# Autodesk Inventor assembly: printer
(part 2 of 2)
- Mate:166: z_motor_mount:2 ↔ CSN 02 1702 B B 4,3:122
- Mate:167: z_motor_mount:2 ↔ CSN 02 1702 B B 4,3:122
- Mate:168: frame:1 ↔ CSN 02 1702 B B 4,3:123
- Mate:169: frame:1 ↔ CSN 02 1702 B B 4,3:123
- Mate:170: frame:1 ↔ CSN 02 1702 B B 4,3:124
- Mate:171: frame:1 ↔ CSN 02 1702 B B 4,3:124
- Mate:172: frame:1 ↔ CSN 02 1702 B B 4,3:117
- Mate:173: frame:1 ↔ CSN 02 1702 B B 4,3:117
- Insert:23: CSN 02 1702 B B 4,3:120 ↔ ISO 4762 M4 x 20:64
- Insert:24: CSN 02 1702 B B 4,3:121 ↔ ISO 4762 M4 x 20:63
- Insert:25: CSN 02 1702 B B 4,3:116 ↔ ISO 4762 M4 x 20:62
- Insert:26: CSN 02 1702 B B 4,3:122 ↔ ISO 4762 M4 x 20:61
- Insert:27: CSN 02 1702 B B 4,3:123 ↔ ISO 4762 M4 x 20:60
- Insert:28: CSN 02 1702 B B 4,3:124 ↔ ISO 4762 M4 x 20:58
- Insert:29: CSN 02 1702 B B 4,3:117 ↔ ISO 4762 M4 x 20:59
- Mate:174: z_motor_brace:2 ↔ CSN 02 1702 B B 4,3:125
- Mate:175: CSN 02 1702 B B 4,3:125 ↔ ISO 4762 M4 x 20:59
- Mate:176: z_motor_brace:2 ↔ CSN 02 1702 B B 4,3:115
- Mate:177: CSN 02 1702 B B 4,3:115 ↔ ISO 4762 M4 x 20:64
- Mate:178: z_rod_stopper_bottom:2 ↔ CSN 02 1702 B B 4,3:119
- Mate:179: CSN 02 1702 B B 4,3:119 ↔ ISO 4762 M4 x 20:63
- Mate:180: z_motor_mount:2 ↔ CSN 02 1702 B B 4,3:128
- Mate:181: CSN 02 1702 B B 4,3:128 ↔ ISO 4762 M4 x 20:60
- Mate:182: z_motor_mount:2 ↔ CSN 02 1702 B B 4,3:118
- Mate:183: CSN 02 1702 B B 4,3:118 ↔ ISO 4762 M4 x 20:58
- Mate:184: brace_right:1 ↔ CSN 02 1702 B B 4,3:126
- Mate:185: CSN 02 1702 B B 4,3:126 ↔ ISO 4762 M4 x 20:62
- Mate:186: z_rod_stopper_bottom:2 ↔ CSN 02 1702 B B 4,3:127
- Mate:187: CSN 02 1702 B B 4,3:127 ↔ ISO 4762 M4 x 20:61
- Mate:188: CSN 02 1702 B B 4,3:119 ↔ DIN EN ISO 7040 M4:51
- Mate:189: ISO 4762 M4 x 20:63 ↔ DIN EN ISO 7040 M4:51
- Mate:190: CSN 02 1702 B B 4,3:115 ↔ DIN EN ISO 7040 M4:54
- Mate:191: ISO 4762 M4 x 20:64 ↔ DIN EN ISO 7040 M4:54
- Mate:192: CSN 02 1702 B B 4,3:125 ↔ DIN EN ISO 7040 M4:52
- Mate:193: ISO 4762 M4 x 20:59 ↔ DIN EN ISO 7040 M4:52
- Mate:194: CSN 02 1702 B B 4,3:128 ↔ DIN EN ISO 7040 M4:53
- Mate:195: ISO 4762 M4 x 20:60 ↔ DIN EN ISO 7040 M4:53
- Mate:196: CSN 02 1702 B B 4,3:118 ↔ DIN EN ISO 7040 M4:55
- Mate:197: ISO 4762 M4 x 20:58 ↔ DIN EN ISO 7040 M4:55
- Mate:198: CSN 02 1702 B B 4,3:126 ↔ DIN EN ISO 7040 M4:50
- Mate:199: ISO 4762 M4 x 20:62 ↔ DIN EN ISO 7040 M4:50
- Mate:200: CSN 02 1702 B B 4,3:127 ↔ DIN EN ISO 7040 M4:49
- Mate:201: ISO 4762 M4 x 20:61 ↔ DIN EN ISO 7040 M4:49
- Mate:202: brace_right:1 ↔ wiring_brace:1
- Mate:203: frame:1 ↔ wiring_brace:1
- Mate:204: brace_right:1 ↔ wiring_brace:1
- Mate:205: brace_left:1 ↔ wiring_brace:2
- Mate:206: frame:1 ↔ wiring_brace:2
- Mate:207: brace_left:1 ↔ wiring_brace:2
- Mate:208: frame:1 ↔ CSN 02 1702 B B 4,3:132
- Mate:209: frame:1 ↔ CSN 02 1702 B B 4,3:132
- Mate:210: wiring_brace:1 ↔ CSN 02 1702 B B 4,3:131
- Mate:211: brace_right:1 ↔ CSN 02 1702 B B 4,3:129
- Mate:212: brace_right:1 ↔ CSN 02 1702 B B 4,3:129
- Mate:213: wiring_brace:1 ↔ CSN 02 1702 B B 4,3:130
- Insert:30: CSN 02 1702 B B 4,3:132 ↔ ISO 4762 M4 x 20:65
- Insert:31: CSN 02 1702 B B 4,3:129 ↔ ISO 4762 M4 x 20:66
- Mate:214: CSN 02 1702 B B 4,3:131 ↔ ISO 4762 M4 x 20:65
- Mate:215: CSN 02 1702 B B 4,3:130 ↔ ISO 4762 M4 x 20:66
- Mate:216: CSN 02 1702 B B 4,3:131 ↔ DIN EN ISO 7040 M4:57
- Mate:217: ISO 4762 M4 x 20:65 ↔ DIN EN ISO 7040 M4:57
- Mate:218: CSN 02 1702 B B 4,3:130 ↔ DIN EN ISO 7040 M4:56
- Mate:219: ISO 4762 M4 x 20:66 ↔ DIN EN ISO 7040 M4:56
- Mate:220: z_motor_mount:2 ↔ CSN 02 1702 B B 3,2:3
- Mate:221: z_motor_mount:2 ↔ CSN 02 1702 B B 3,2:2
- Mate:222: z_motor_mount:2 ↔ CSN 02 1702 B B 3,2:1
- Mate:223: z_motor_mount:2 ↔ CSN 02 1702 B B 3,2:4
- Mate:224: z_motor_mount:2 ↔ CSN 02 1702 B B 3,2:2
- Mate:225: z_motor_mount:2 ↔ CSN 02 1702 B B 3,2:4
- Mate:226: z_motor_mount:2 ↔ CSN 02 1702 B B 3,2:3
- Mate:227: z_motor_mount:2 ↔ CSN 02 1702 B B 3,2:1
- Insert:32: CSN 02 1702 B B 3,2:4 ↔ ISO 4762 M3 x 16:2
- Insert:33: CSN 02 1702 B B 3,2:2 ↔ ISO 4762 M3 x 16:1
- Insert:34: CSN 02 1702 B B 3,2:3 ↔ ISO 4762 M3 x 16:3
- Insert:35: CSN 02 1702 B B 3,2:1 ↔ ISO 4762 M3 x 16:4
- Mate:228: CSN 02 1702 B B 4,3:136 ↔ ISO 4762 M4 x 20:67
- Insert:36: CSN 02 1702 B B 4,3:142 ↔ ISO 4762 M4 x 20:67
- Mate:229: CSN 02 1702 B B 4,3:143 ↔ ISO 4762 M4 x 20:68
- Insert:37: CSN 02 1702 B B 4,3:135 ↔ ISO 4762 M4 x 20:68
- Mate:230: CSN 02 1702 B B 4,3:146 ↔ ISO 4762 M4 x 20:69
- Insert:38: CSN 02 1702 B B 4,3:141 ↔ ISO 4762 M4 x 20:69
- Mate:231: CSN 02 1702 B B 4,3:145 ↔ ISO 4762 M4 x 20:70
- Insert:39: CSN 02 1702 B B 4,3:140 ↔ ISO 4762 M4 x 20:70
- Mate:232: CSN 02 1702 B B 4,3:144 ↔ ISO 4762 M4 x 20:71
- Insert:40: CSN 02 1702 B B 4,3:134 ↔ ISO 4762 M4 x 20:71
- Mate:233: CSN 02 1702 B B 4,3:137 ↔ ISO 4762 M4 x 20:72
- Insert:41: CSN 02 1702 B B 4,3:139 ↔ ISO 4762 M4 x 20:72
- Mate:234: CSN 02 1702 B B 4,3:133 ↔ ISO 4762 M4 x 20:73
- Insert:42: CSN 02 1702 B B 4,3:138 ↔ ISO 4762 M4 x 20:73
- Mate:235: ISO 4762 M4 x 20:70 ↔ DIN EN ISO 7040 M4:58
- Mate:236: CSN 02 1702 B B 4,3:145 ↔ DIN EN ISO 7040 M4:58
- Mate:237: ISO 4762 M4 x 20:71 ↔ DIN EN ISO 7040 M4:59
- Mate:238: CSN 02 1702 B B 4,3:144 ↔ DIN EN ISO 7040 M4:59
- Mate:239: ISO 4762 M4 x 20:72 ↔ DIN EN ISO 7040 M4:60
- Mate:240: CSN 02 1702 B B 4,3:137 ↔ DIN EN ISO 7040 M4:60
- Mate:241: ISO 4762 M4 x 20:68 ↔ DIN EN ISO 7040 M4:61
- Mate:242: CSN 02 1702 B B 4,3:143 ↔ DIN EN ISO 7040 M4:61
- Mate:243: ISO 4762 M4 x 20:69 ↔ DIN EN ISO 7040 M4:62
- Mate:244: CSN 02 1702 B B 4,3:146 ↔ DIN EN ISO 7040 M4:62
- Mate:245: ISO 4762 M4 x 20:73 ↔ DIN EN ISO 7040 M4:63
- Mate:246: CSN 02 1702 B B 4,3:133 ↔ DIN EN ISO 7040 M4:63
- Mate:247: ISO 4762 M4 x 20:67 ↔ DIN EN ISO 7040 M4:64
- Mate:248: CSN 02 1702 B B 4,3:136 ↔ DIN EN ISO 7040 M4:64
- Mate:249: CSN 02 1702 B B 4,3:149 ↔ ISO 4762 M4 x 20:74
- Insert:43: CSN 02 1702 B B 4,3:150 ↔ ISO 4762 M4 x 20:74
- Mate:250: CSN 02 1702 B B 4,3:148 ↔ ISO 4762 M4 x 20:75
- Insert:44: CSN 02 1702 B B 4,3:147 ↔ ISO 4762 M4 x 20:75
- Mate:251: ISO 4762 M4 x 20:75 ↔ DIN EN ISO 7040 M4:65
- Mate:252: CSN 02 1702 B B 4,3:148 ↔ DIN EN ISO 7040 M4:65
- Mate:253: ISO 4762 M4 x 20:74 ↔ DIN EN ISO 7040 M4:66
- Mate:254: CSN 02 1702 B B 4,3:149 ↔ DIN EN ISO 7040 M4:66
- Insert:45: CSN 02 1702 B B 3,2:6 ↔ ISO 4762 M3 x 16:5
- Insert:46: CSN 02 1702 B B 3,2:8 ↔ ISO 4762 M3 x 16:6
- Insert:47: CSN 02 1702 B B 3,2:7 ↔ ISO 4762 M3 x 16:7
- Insert:48: CSN 02 1702 B B 3,2:5 ↔ ISO 4762 M3 x 16:8
- Mate:255: back:1 ↔ PC Fan:1
- Mate:256: back:1 ↔ PC Fan:1
- Mate:257: back:1 ↔ PC Fan:1
- Mate:258 (3 mm): back:1 ↔ User Library-Fan Guard:1
- Mate:259: y_carriage_belt_iddler:2 ↔ y_carriage_belt_iddler_holder:1
- Mate:260: y_carriage_belt_iddler:2 ↔ y_carriage_belt_iddler_holder:1
- Mate:261: y_carriage_belt_iddler:2 ↔ y_carriage_belt_iddler_holder:1
- Mate:262: y_carriage_belt_iddler:1 ↔ y_carriage_belt_iddler_holder:1
- Mate:263: y_carriage_belt_iddler:1 ↔ y_carriage_belt_iddler_holder:1
- Mate:264: y_carriage_belt_iddler:1 ↔ y_carriage_belt_iddler_holder:1
- Mate:265: 608RS:1 ↔ belt_guide:1
- Mate:266: 608RS:1 ↔ belt_guide:1
- Mate:267: belt_guide:1 ↔ belt_guide:2
- Mate:268: belt_guide:1 ↔ belt_guide:2
- Mate:269: 608RS:1 ↔ belt_guide:2
- Mate:270: CSN 02 1702 B B 8,4:5 ↔ CSN 02 1702 B B 8,4:6
- Mate:271: CSN 02 1702 B B 8,4:5 ↔ CSN 02 1702 B B 8,4:6
- Mate:272: CSN 02 1702 B B 8,4:3 ↔ CSN 02 1702 B B 8,4:4
- Mate:273: CSN 02 1702 B B 8,4:3 ↔ CSN 02 1702 B B 8,4:4
- Mate:274: 608RS:1 ↔ CSN 02 1702 B B 8,4:4
- Mate:275: 608RS:1 ↔ CSN 02 1702 B B 8,4:4
- Mate:276: 608RS:1 ↔ CSN 02 1702 B B 8,4:5
- Mate:277: 608RS:1 ↔ CSN 02 1702 B B 8,4:5
- Mate:278: y_carriage_belt_iddler:1 ↔ CSN 02 1702 B B 8,4:6
- Mate:279: y_carriage_belt_iddler:2 ↔ 608RS:1
- Mate:280: y_carriage_belt_iddler:2 ↔ CSN 02 1702 B B 8,4:1
- Mate:281: y_carriage_belt_iddler:2 ↔ CSN 02 1702 B B 8,4:1
- Mate:282: y_carriage_belt_iddler:1 ↔ CSN 02 1702 B B 8,4:2
- Mate:283: y_carriage_belt_iddler:1 ↔ CSN 02 1702 B B 8,4:2
- Insert:49: CSN 02 1702 B B 8,4:2 ↔ ISO 4762 M8 x 40:1
- Mate:284: CSN 02 1702 B B 8,4:1 ↔ DIN EN ISO 7040 M8:1
- Mate:285: ISO 4762 M8 x 40:1 ↔ DIN EN ISO 7040 M8:1
- Mate:286: back:1 ↔ y_carriage_belt_iddler:2
- Mate:287: back:1 ↔ y_carriage_belt_iddler:2
- Mate:288: back:1 ↔ y_carriage_belt_iddler:1
- Mate:289: back:1 ↔ CSN 02 1702 B B 4,3:152
- Mate:290: back:1 ↔ CSN 02 1702 B B 4,3:153
- Mate:291: back:1 ↔ CSN 02 1702 B B 4,3:153
- Mate:292: back:1 ↔ CSN 02 1702 B B 4,3:152
- Insert:50: CSN 02 1702 B B 4,3:152 ↔ ISO 4762 M4 x 30:1
- Insert:51: CSN 02 1702 B B 4,3:153 ↔ ISO 4762 M4 x 30:2
- Mate:293: y_carriage_belt_iddler_holder:1 ↔ CSN 02 1702 B B 4,3:154
- Mate:294: y_carriage_belt_iddler_holder:1 ↔ CSN 02 1702 B B 4,3:151
- Mate:295: CSN 02 1702 B B 4,3:151 ↔ ISO 4762 M4 x 30:2
- Mate:296: CSN 02 1702 B B 4,3:154 ↔ ISO 4762 M4 x 30:1
- Mate:297: CSN 02 1702 B B 4,3:151 ↔ DIN EN ISO 7040 M4:68
- Mate:298: ISO 4762 M4 x 30:2 ↔ DIN EN ISO 7040 M4:68
- Mate:299: CSN 02 1702 B B 4,3:154 ↔ DIN EN ISO 7040 M4:67
- Mate:300: ISO 4762 M4 x 30:1 ↔ DIN EN ISO 7040 M4:67
- Mate:301: y_motor_mount:1 ↔ y_motor_mount_brace:1
- Mate:302: y_motor_mount:1 ↔ y_motor_mount_brace:1
- Mate:303: y_motor_mount:1 ↔ y_motor_mount_brace:1
- Mate:304: front:1 ↔ y_motor_mount:1
- Mate:305: front:1 ↔ y_motor_mount_brace:1
- Mate:306: front:1 ↔ y_motor_mount:1
- Mate:307: front:1 ↔ CSN 02 1702 B B 4,3:159
- Mate:308: front:1 ↔ CSN 02 1702 B B 4,3:160
- Mate:309: front:1 ↔ CSN 02 1702 B B 4,3:160
- Mate:310: front:1 ↔ CSN 02 1702 B B 4,3:159
- Mate:311: y_motor_mount:1 ↔ CSN 02 1702 B B 4,3:157
- Mate:312: y_motor_mount:1 ↔ CSN 02 1702 B B 4,3:157
- Insert:52: CSN 02 1702 B B 4,3:160 ↔ ISO 4762 M4 x 20:78
- Insert:53: CSN 02 1702 B B 4,3:159 ↔ ISO 4762 M4 x 20:77
- Insert:54: CSN 02 1702 B B 4,3:157 ↔ ISO 4762 M4 x 20:76
- Mate:313: y_motor_mount_brace:1 ↔ CSN 02 1702 B B 4,3:158
- Mate:314: CSN 02 1702 B B 4,3:158 ↔ ISO 4762 M4 x 20:78
- Mate:315: y_motor_mount_brace:1 ↔ CSN 02 1702 B B 4,3:155
- Mate:316: CSN 02 1702 B B 4,3:155 ↔ ISO 4762 M4 x 20:76
- Mate:317: y_motor_mount:1 ↔ CSN 02 1702 B B 4,3:156
- Mate:318: CSN 02 1702 B B 4,3:156 ↔ ISO 4762 M4 x 20:77
- Mate:319: CSN 02 1702 B B 4,3:156 ↔ DIN EN ISO 7040 M4:70
- Mate:320: ISO 4762 M4 x 20:77 ↔ DIN EN ISO 7040 M4:70
- Mate:321: CSN 02 1702 B B 4,3:158 ↔ DIN EN ISO 7040 M4:69
- Mate:322: ISO 4762 M4 x 20:78 ↔ DIN EN ISO 7040 M4:69
- Mate:323: CSN 02 1702 B B 4,3:155 ↔ DIN EN ISO 7040 M4:71
- Mate:324: ISO 4762 M4 x 20:76 ↔ DIN EN ISO 7040 M4:71
- Mate:325: motor_spacer:1 ↔ NEMA 17 with T5 Pulley:1
- Mate:326: motor_spacer:1 ↔ NEMA 17 with T5 Pulley:1
- Mate:327: motor_spacer:1 ↔ NEMA 17 with T5 Pulley:1
- Mate:328: y_motor_mount:1 ↔ motor_spacer:1
- Tangent:1: y_motor_mount:1 ↔ motor_spacer:1
- Tangent:2: y_motor_mount:1 ↔ motor_spacer:1
- Mate:329: y_motor_mount:1 ↔ CSN 02 1702 B B 3,2:12
- Mate:330: y_motor_mount:1 ↔ CSN 02 1702 B B 3,2:11
- Mate:331: y_motor_mount:1 ↔ CSN 02 1702 B B 3,2:9
- Mate:332: y_motor_mount:1 ↔ CSN 02 1702 B B 3,2:10
- Insert:55: CSN 02 1702 B B 3,2:12 ↔ ISO 4762 M3 x 16:12
- Insert:56: CSN 02 1702 B B 3,2:11 ↔ ISO 4762 M3 x 16:11
- Insert:57: CSN 02 1702 B B 3,2:9 ↔ ISO 4762 M3 x 16:10
- Insert:58: CSN 02 1702 B B 3,2:10 ↔ ISO 4762 M3 x 16:9
- Mate:333: motor_spacer:1 ↔ ISO 4762 M3 x 16:12
- Mate:334: motor_spacer:1 ↔ ISO 4762 M3 x 16:11
- Mate:335: motor_spacer:1 ↔ ISO 4762 M3 x 16:9
- Mate:336: motor_spacer:1 ↔ ISO 4762 M3 x 16:10
- Mate:337: y_axis_rod:2 ↔ y_carryage:1
- Mate:338: y_axis_rod:1 ↔ y_carryage:1
- Mate:339: z_axis_rod:2 ↔ x_axis:1
- Mate:340: z_axis_rod:1 ↔ x_axis:1
- Mate:341: brace_right:1 ↔ CSN 02 1702 B B 4,3:161
- Mate:342: brace_right:1 ↔ CSN 02 1702 B B 4,3:161
- Insert:59: CSN 02 1702 B B 4,3:161 ↔ ISO 4762 M4 x 20:79
- Mate:343: frame_brace_top:1 ↔ CSN 02 1702 B B 4,3:162
- Mate:344: CSN 02 1702 B B 4,3:162 ↔ ISO 4762 M4 x 20:79
- Mate:345: CSN 02 1702 B B 4,3:162 ↔ DIN EN ISO 7040 M4:72
- Mate:346: ISO 4762 M4 x 20:79 ↔ DIN EN ISO 7040 M4:72
- Mate:347: CSN 02 1702 B B 4,3:164 ↔ ISO 4762 M4 x 20:80
- Insert:60: CSN 02 1702 B B 4,3:163 ↔ ISO 4762 M4 x 20:80
- Mate:348: ISO 4762 M4 x 20:80 ↔ DIN EN ISO 7040 M4:73
- Mate:349: CSN 02 1702 B B 4,3:164 ↔ DIN EN ISO 7040 M4:73
- Mate:350: z_axis_top_cap:2 ↔ CSN 02 1702 B B 4,3:172
- Mate:351: z_axis_top_cap:2 ↔ CSN 02 1702 B B 4,3:174
- Mate:352: z_axis_top_cap:2 ↔ CSN 02 1702 B B 4,3:174
- Mate:353: z_axis_top_cap:2 ↔ CSN 02 1702 B B 4,3:172
- Mate:354: z_axis_top:2 ↔ CSN 02 1702 B B 4,3:173
- Mate:355: z_axis_top:2 ↔ CSN 02 1702 B B 4,3:171
- Mate:356: z_axis_top:2 ↔ CSN 02 1702 B B 4,3:170
- Mate:357: z_axis_top:2 ↔ CSN 02 1702 B B 4,3:170
- Mate:358: z_axis_top:2 ↔ CSN 02 1702 B B 4,3:173
- Mate:359: z_axis_top:2 ↔ CSN 02 1702 B B 4,3:171
- Insert:61: CSN 02 1702 B B 4,3:170 ↔ ISO 4762 M4 x 20:81
- Insert:62: CSN 02 1702 B B 4,3:171 ↔ ISO 4762 M4 x 20:82
- Insert:63: CSN 02 1702 B B 4,3:173 ↔ ISO 4762 M4 x 20:83
- Insert:64: CSN 02 1702 B B 4,3:174 ↔ ISO 4762 M4 x 20:84
- Insert:65: CSN 02 1702 B B 4,3:172 ↔ ISO 4762 M4 x 20:85
- Mate:360: brace_right:1 ↔ CSN 02 1702 B B 4,3:169
- Mate:361: CSN 02 1702 B B 4,3:169 ↔ ISO 4762 M4 x 20:81
- Mate:362: frame:1 ↔ CSN 02 1702 B B 4,3:165
- Mate:363: CSN 02 1702 B B 4,3:165 ↔ ISO 4762 M4 x 20:83
- Mate:364: frame:1 ↔ CSN 02 1702 B B 4,3:166
- Mate:365: CSN 02 1702 B B 4,3:166 ↔ ISO 4762 M4 x 20:82
- Mate:366: z_axis_top:2 ↔ CSN 02 1702 B B 4,3:167
- Mate:367: CSN 02 1702 B B 4,3:167 ↔ ISO 4762 M4 x 20:84
- Mate:368: z_axis_top:2 ↔ CSN 02 1702 B B 4,3:168
- Mate:369: CSN 02 1702 B B 4,3:169 ↔ DIN EN ISO 7040 M4:78
- Mate:370: ISO 4762 M4 x 20:81 ↔ DIN EN ISO 7040 M4:78
- Mate:371: CSN 02 1702 B B 4,3:166 ↔ DIN EN ISO 7040 M4:77
- Mate:372: ISO 4762 M4 x 20:82 ↔ DIN EN ISO 7040 M4:77
- Mate:373: CSN 02 1702 B B 4,3:165 ↔ DIN EN ISO 7040 M4:76
- Mate:374: ISO 4762 M4 x 20:83 ↔ DIN EN ISO 7040 M4:76
- Mate:375: CSN 02 1702 B B 4,3:167 ↔ DIN EN ISO 7040 M4:75
- Mate:376: ISO 4762 M4 x 20:84 ↔ DIN EN ISO 7040 M4:75
- Mate:377: CSN 02 1702 B B 4,3:168 ↔ DIN EN ISO 7040 M4:74
- Mate:378: CSN 02 1702 B B 4,3:168 ↔ ISO 4762 M4 x 20:85
- Mate:379: ISO 4762 M4 x 20:85 ↔ DIN EN ISO 7040 M4:74
- Mate:380: CSN 02 1702 B B 4,3:179 ↔ ISO 4762 M4 x 20:86
- Insert:66: CSN 02 1702 B B 4,3:180 ↔ ISO 4762 M4 x 20:86
- Mate:381: CSN 02 1702 B B 4,3:176 ↔ ISO 4762 M4 x 20:87
- Insert:67: CSN 02 1702 B B 4,3:181 ↔ ISO 4762 M4 x 20:87
- Mate:382: CSN 02 1702 B B 4,3:175 ↔ ISO 4762 M4 x 20:88
- Insert:68: CSN 02 1702 B B 4,3:183 ↔ ISO 4762 M4 x 20:88
- Mate:383: CSN 02 1702 B B 4,3:177 ↔ ISO 4762 M4 x 20:89
- Insert:69: CSN 02 1702 B B 4,3:184 ↔ ISO 4762 M4 x 20:89
- Mate:384: CSN 02 1702 B B 4,3:178 ↔ ISO 4762 M4 x 20:90
- Insert:70: CSN 02 1702 B B 4,3:182 ↔ ISO 4762 M4 x 20:90
- Mate:385: ISO 4762 M4 x 20:90 ↔ DIN EN ISO 7040 M4:79
- Mate:386: CSN 02 1702 B B 4,3:178 ↔ DIN EN ISO 7040 M4:79
- Mate:387: ISO 4762 M4 x 20:89 ↔ DIN EN ISO 7040 M4:80
- Mate:388: CSN 02 1702 B B 4,3:177 ↔ DIN EN ISO 7040 M4:80
- Mate:389: ISO 4762 M4 x 20:88 ↔ DIN EN ISO 7040 M4:81
- Mate:390: CSN 02 1702 B B 4,3:175 ↔ DIN EN ISO 7040 M4:81
- Mate:391: ISO 4762 M4 x 20:87 ↔ DIN EN ISO 7040 M4:82
- Mate:392: CSN 02 1702 B B 4,3:176 ↔ DIN EN ISO 7040 M4:82
- Mate:393: ISO 4762 M4 x 20:86 ↔ DIN EN ISO 7040 M4:83
- Mate:394: CSN 02 1702 B B 4,3:179 ↔ DIN EN ISO 7040 M4:83
- Mate:402: front:1 ↔ front_panel_2004_brace_left:1
- Mate:403: front:1 ↔ front_panel_2004_brace_left:1
- Flush:7: front:1 ↔ front_panel_2004_brace_left:1
- Flush:8: lcd:1 ↔ front_panel_2004_display:1
- Mate:404: lcd:1 ↔ front_panel_2004_display:1
- Mate:405: lcd:1 ↔ front_panel_2004_display:1
- Mate:406: front_panel_2004_brace_left:1 ↔ front_panel_2004_display:1
- Mate:407: front_panel_2004_brace_left:1 ↔ front_panel_2004_display:1
- Mate:408: front_panel_2004_brace_left:1 ↔ front_panel_2004_display:1
- Mate:409: front_panel_2004_brace_left:1 ↔ front_panel_2004_front:1
- Mate:410: front_panel_2004_brace_left:1 ↔ front_panel_2004_front:1
- Mate:411: front_panel_2004_brace_left:1 ↔ front_panel_2004_front:1
- Mate:412: front_panel_2004_brace_left:1 ↔ front_panel_2004_bottom:1
- Mate:413: front_panel_2004_brace_left:1 ↔ front_panel_2004_bottom:1
- Mate:414: front_panel_2004_brace_left:1 ↔ front_panel_2004_bottom:1
- Mate:415: front:1 ↔ front_panel_2004_brace_right:1
- Mate:416: front_panel_2004_display:1 ↔ front_panel_2004_brace_right:1
- Mate:417: front_panel_2004_display:1 ↔ front_panel_2004_brace_right:1
- Mate:418: front_panel_2004_brace_right:1 ↔ CSN 02 1702 B B 4,3:199
- Mate:419: front_panel_2004_brace_right:1 ↔ CSN 02 1702 B B 4,3:199
- Mate:420: front_panel_2004_brace_right:1 ↔ CSN 02 1702 B B 4,3:200
- Mate:421: front_panel_2004_brace_right:1 ↔ CSN 02 1702 B B 4,3:200
- Mate:422: front_panel_2004_brace_right:1 ↔ CSN 02 1702 B B 4,3:198
- Mate:423: front_panel_2004_brace_right:1 ↔ CSN 02 1702 B B 4,3:198
- Mate:424: front_panel_2004_brace_right:1 ↔ CSN 02 1702 B B 4,3:197
- Mate:425: front_panel_2004_brace_right:1 ↔ CSN 02 1702 B B 4,3:197
- Mate:426: front_panel_2004_brace_right:1 ↔ CSN 02 1702 B B 4,3:196
- Mate:427: front_panel_2004_brace_right:1 ↔ CSN 02 1702 B B 4,3:196
- Mate:428: front_panel_2004_brace_right:1 ↔ CSN 02 1702 B B 4,3:195
- Mate:429: front_panel_2004_brace_right:1 ↔ CSN 02 1702 B B 4,3:195
- Mate:430: front:1 ↔ CSN 02 1702 B B 4,3:194
- Mate:431: front:1 ↔ CSN 02 1702 B B 4,3:194
- Mate:432: front:1 ↔ CSN 02 1702 B B 4,3:186
- Mate:433: front:1 ↔ CSN 02 1702 B B 4,3:186
- Insert:71: CSN 02 1702 B B 4,3:197 ↔ ISO 4762 M4 x 20:91
- Insert:72: CSN 02 1702 B B 4,3:199 ↔ ISO 4762 M4 x 20:98
- Insert:73: CSN 02 1702 B B 4,3:196 ↔ ISO 4762 M4 x 20:97
- Insert:74: CSN 02 1702 B B 4,3:195 ↔ ISO 4762 M4 x 20:92
- Insert:75: CSN 02 1702 B B 4,3:200 ↔ ISO 4762 M4 x 20:93
- Insert:76: CSN 02 1702 B B 4,3:198 ↔ ISO 4762 M4 x 20:94
- Insert:77: CSN 02 1702 B B 4,3:186 ↔ ISO 4762 M4 x 20:95
- Insert:78: CSN 02 1702 B B 4,3:194 ↔ ISO 4762 M4 x 20:96
- Mate:434: front_panel_2004_display:1 ↔ CSN 02 1702 B B 4,3:193
- Mate:435: CSN 02 1702 B B 4,3:193 ↔ ISO 4762 M4 x 20:94
- Mate:436: front_panel_2004_display:1 ↔ CSN 02 1702 B B 4,3:187
- Mate:437: CSN 02 1702 B B 4,3:187 ↔ ISO 4762 M4 x 20:93
- Mate:438: front_panel_2004_display:1 ↔ CSN 02 1702 B B 4,3:188
- Mate:439: CSN 02 1702 B B 4,3:188 ↔ ISO 4762 M4 x 20:98
- Mate:440: front_panel_2004_front:1 ↔ CSN 02 1702 B B 4,3:185
- Mate:441: CSN 02 1702 B B 4,3:185 ↔ ISO 4762 M4 x 20:91
- Mate:442: front_panel_2004_brace_right:1 ↔ CSN 02 1702 B B 4,3:192
- Mate:443: CSN 02 1702 B B 4,3:192 ↔ ISO 4762 M4 x 20:96
- Mate:444: front_panel_2004_brace_right:1 ↔ CSN 02 1702 B B 4,3:189
- Mate:445: CSN 02 1702 B B 4,3:189 ↔ ISO 4762 M4 x 20:95
- Mate:446: front_panel_2004_bottom:1 ↔ CSN 02 1702 B B 4,3:191
- Mate:447: CSN 02 1702 B B 4,3:191 ↔ ISO 4762 M4 x 20:97
- Mate:448: front_panel_2004_bottom:1 ↔ CSN 02 1702 B B 4,3:190
- Mate:449: CSN 02 1702 B B 4,3:190 ↔ ISO 4762 M4 x 20:92
- Mate:450: CSN 02 1702 B B 4,3:190 ↔ DIN EN ISO 7040 M4:91
- Mate:451: ISO 4762 M4 x 20:92 ↔ DIN EN ISO 7040 M4:91
- Mate:452: CSN 02 1702 B B 4,3:191 ↔ DIN EN ISO 7040 M4:85
- Mate:453: ISO 4762 M4 x 20:97 ↔ DIN EN ISO 7040 M4:85
- Mate:454: CSN 02 1702 B B 4,3:185 ↔ DIN EN ISO 7040 M4:84
- Mate:455: ISO 4762 M4 x 20:91 ↔ DIN EN ISO 7040 M4:84
- Mate:456: CSN 02 1702 B B 4,3:188 ↔ DIN EN ISO 7040 M4:90
- Mate:457: ISO 4762 M4 x 20:98 ↔ DIN EN ISO 7040 M4:90
- Mate:458: CSN 02 1702 B B 4,3:187 ↔ DIN EN ISO 7040 M4:89
- Mate:459: ISO 4762 M4 x 20:93 ↔ DIN EN ISO 7040 M4:89
- Mate:460: CSN 02 1702 B B 4,3:193 ↔ DIN EN ISO 7040 M4:86
- Mate:461: ISO 4762 M4 x 20:94 ↔ DIN EN ISO 7040 M4:86
- Mate:462: CSN 02 1702 B B 4,3:192 ↔ DIN EN ISO 7040 M4:87
- Mate:463: ISO 4762 M4 x 20:96 ↔ DIN EN ISO 7040 M4:87
- Mate:464: CSN 02 1702 B B 4,3:189 ↔ DIN EN ISO 7040 M4:88
- Mate:465: ISO 4762 M4 x 20:95 ↔ DIN EN ISO 7040 M4:88
- Mate:466: CSN 02 1702 B B 4,3:201 ↔ ISO 4762 M4 x 20:99
- Insert:79: CSN 02 1702 B B 4,3:211 ↔ ISO 4762 M4 x 20:99
- Mate:467: CSN 02 1702 B B 4,3:205 ↔ ISO 4762 M4 x 20:100
- Insert:80: CSN 02 1702 B B 4,3:209 ↔ ISO 4762 M4 x 20:100
- Mate:468: CSN 02 1702 B B 4,3:204 ↔ ISO 4762 M4 x 20:101
- Insert:81: CSN 02 1702 B B 4,3:202 ↔ ISO 4762 M4 x 20:101
- Mate:469: CSN 02 1702 B B 4,3:207 ↔ ISO 4762 M4 x 20:102
- Insert:82: CSN 02 1702 B B 4,3:208 ↔ ISO 4762 M4 x 20:102
- Mate:470: CSN 02 1702 B B 4,3:206 ↔ ISO 4762 M4 x 20:103
- Insert:83: CSN 02 1702 B B 4,3:210 ↔ ISO 4762 M4 x 20:103
- Mate:471: CSN 02 1702 B B 4,3:203 ↔ ISO 4762 M4 x 20:104
- Insert:84: CSN 02 1702 B B 4,3:212 ↔ ISO 4762 M4 x 20:104
- Mate:472: ISO 4762 M4 x 20:99 ↔ DIN EN ISO 7040 M4:92
- Mate:473: CSN 02 1702 B B 4,3:201 ↔ DIN EN ISO 7040 M4:92
- Mate:474: ISO 4762 M4 x 20:103 ↔ DIN EN ISO 7040 M4:93
- Mate:475: CSN 02 1702 B B 4,3:206 ↔ DIN EN ISO 7040 M4:93
- Mate:476: ISO 4762 M4 x 20:102 ↔ DIN EN ISO 7040 M4:94
- Mate:477: CSN 02 1702 B B 4,3:207 ↔ DIN EN ISO 7040 M4:94
- Mate:478: ISO 4762 M4 x 20:101 ↔ DIN EN ISO 7040 M4:95
- Mate:479: CSN 02 1702 B B 4,3:204 ↔ DIN EN ISO 7040 M4:95
- Mate:480: ISO 4762 M4 x 20:104 ↔ DIN EN ISO 7040 M4:96
- Mate:481: CSN 02 1702 B B 4,3:203 ↔ DIN EN ISO 7040 M4:96
- Mate:482: ISO 4762 M4 x 20:100 ↔ DIN EN ISO 7040 M4:97
- Mate:483: CSN 02 1702 B B 4,3:205 ↔ DIN EN ISO 7040 M4:97
- Mate:484: bottom:1 ↔ CSN 02 1702 B B 4,3:213
- Mate:485: bottom:1 ↔ CSN 02 1702 B B 4,3:213
- Insert:85: CSN 02 1702 B B 4,3:213 ↔ ISO 4762 M4 x 20:105
- Mate:486: y_motor_mount:1 ↔ CSN 02 1702 B B 4,3:214
- Mate:487: CSN 02 1702 B B 4,3:214 ↔ ISO 4762 M4 x 20:105
- Mate:488: CSN 02 1702 B B 4,3:214 ↔ DIN EN ISO 7040 M4:98
- Mate:489: ISO 4762 M4 x 20:105 ↔ DIN EN ISO 7040 M4:98
- Mate:490: front_panel_2004_front:1 ↔ USB-Socket:1
- Mate:491: front_panel_2004_front:1 ↔ USB-Socket:2
- Mate:492 (0.5 mm): front_panel_2004_front:1 ↔ USB-Socket:1
- Mate:493 (0.5 mm): front_panel_2004_front:1 ↔ USB-Socket:2
- Mate:494 (0.5 mm): front_panel_2004_front:1 ↔ USB-Socket:2
- Mate:495 (0.5 mm): front_panel_2004_front:1 ↔ USB-Socket:1
